# Autodesk Inventor assembly: СБ_Короб задний
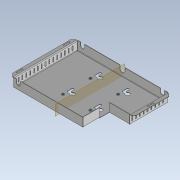
[picture p0: Inventor's stored thumbnail of the model, 180x180]
Saved by Autodesk Inventor 2021.2 (Build 252289000, 289)
## iProperties
Created: 2022-12-06
Part Number: СБ_Короб задний
Document SubType Name: Assembly
Designer: Voodoo
Mass: 154.56 g
Surface Area: 2111.46 cm^2
Volume: 154.56 cm^3
Density: 1 g/cm^3
Author: Voodoo
## Documents named in this file (3)
- C:\Users\Voodoo\Documents\Inventor\АБТ_Инфотабло\СБ_Короб задний.iam
- C:\Users\Voodoo\Documents\Inventor\АБТ_Инфотабло\Короб задний.ipt
- C:\Users\Voodoo\Documents\Inventor\Content Center Files\R2021\Metizi\PEM_S_M5_1.ipt
## Components (5 placed, 2 different names)
1. Короб задний:1
2. PEM_S_M5_1:1
3. PEM_S_M5_1:2
4. PEM_S_M5_1:3
5. PEM_S_M5_1:4
## Relationships (4: Insert 4)
- [Insert]: Короб задний:1 ↔ PEM_S_M5_1:3
- [Insert]: Короб задний:1 ↔ PEM_S_M5_1:2
- [Insert]: Короб задний:1 ↔ PEM_S_M5_1:1
- [Insert]: Короб задний:1 ↔ PEM_S_M5_1:4
